# Autodesk Inventor assembly: zmotorblock(right)
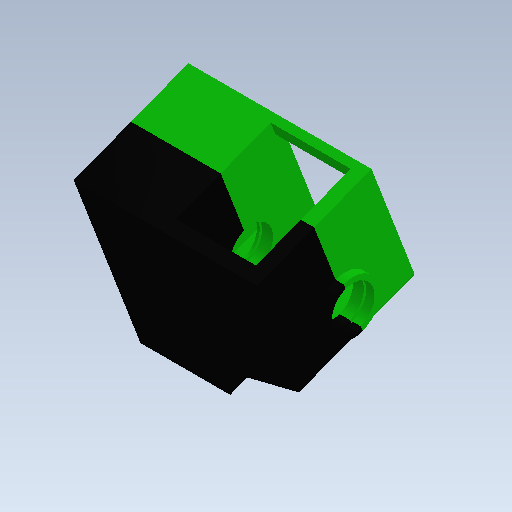
[picture p0: Inventor's stored thumbnail of the model, 512x512]
Saved by Autodesk Inventor 2020.4 (Build 244396000, 396)
## iProperties
Created: 2021-03-29
Part Number: zmotorblock(right)
Document SubType Name: Assembly
Designer: AOB
Mass: 76.5093 g
Surface Area: 348.693 cm^2
Volume: 72.1786 cm^3
Density: 1.06 g/cm^3
Author: AOB
## Documents named in this file (3)
- C:\Users\marti\Documents\Inventor\ProjectBoron\Boron Ultima\zmotorblock(right).iam
- C:\Users\marti\Documents\Inventor\ProjectBoron\Boron Ultima\zmotorblockleft-half(right).ipt
- C:\Users\marti\Documents\Inventor\ProjectBoron\Boron Ultima\zmotorblockright-half(right).ipt
## Components (2 placed, 2 different names)
1. zmotorblockleft-half(right):1 — Rigid:1
2. zmotorblockright-half(right):1 — Rigid:1
## Relationships (1: WeldJoint 1)
- Rigid:1 [WeldJoint]: zmotorblockleft-half(right):1 ↔ zmotorblockright-half(right):1
